# Autodesk Inventor assembly: legAssembly
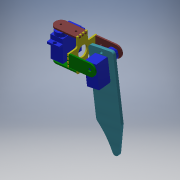
[picture p0: Inventor's stored thumbnail of the model, 180x180]
Saved by Autodesk Inventor 2019.1 (Build 231200000, 200)
## iProperties
Created: 2018-12-04
Part Number: legAssembly
Document SubType Name: Assembly
Designer: kfortuna
Author: kfortuna
## Documents named in this file (6)
- C:\Users\kfortuna\Desktop\legAssembly.iam
- C:\Users\kfortuna\Desktop\Connection4.ipt
- C:\Users\kfortuna\Desktop\cross.ipt
- C:\Users\kfortuna\Desktop\Connection4-3.5.ipt
- C:\Users\kfortuna\Desktop\Servo.ipt
- C:\Users\kfortuna\Desktop\legRound.ipt
## Components (8 placed, 5 different names)
1. Connection4:1 — Mate:1, Mate:2, Flush:1, Insert:1
2. cross:1 — Mate:1, Mate:2, Flush:1, Mate:3, Flush:2, Mate:4, Mate:5, Mate:6, Flush:3, Mate:7, Mate:8, Flush:4
3. Connection4-3.5:1 — Mate:3, Flush:2, Mate:4
4. Connection4:2 — Mate:5, Mate:6, Flush:3, Mate:10, Insert:3
5. Connection4-3.5:2 — Mate:7, Mate:8, Flush:4
6. Servo:1 — Insert:1
7. legRound:1 — Mate:9, Insert:2
8. Servo:2 — Mate:9, Insert:2, Mate:10, Insert:3
## Relationships (17: Mate 10, Flush 4, Insert 3)
- Mate:1: Connection4:1 ↔ cross:1
- Mate:2: Connection4:1 ↔ cross:1
- Flush:1: Connection4:1 ↔ cross:1
- Mate:3: cross:1 ↔ Connection4-3.5:1
- Flush:2: cross:1 ↔ Connection4-3.5:1
- Mate:4: cross:1 ↔ Connection4-3.5:1
- Mate:5: cross:1 ↔ Connection4:2
- Mate:6: cross:1 ↔ Connection4:2
- Flush:3: cross:1 ↔ Connection4:2
- Mate:7: cross:1 ↔ Connection4-3.5:2
- Mate:8: cross:1 ↔ Connection4-3.5:2
- Flush:4: cross:1 ↔ Connection4-3.5:2
- Insert:1: Connection4:1 ↔ Servo:1
- Mate:9: legRound:1 ↔ Servo:2
- Insert:2: legRound:1 ↔ Servo:2
- Mate:10: Connection4:2 ↔ Servo:2
- Insert:3: Connection4:2 ↔ Servo:2
